# Autodesk Inventor assembly: BBM - Simplified
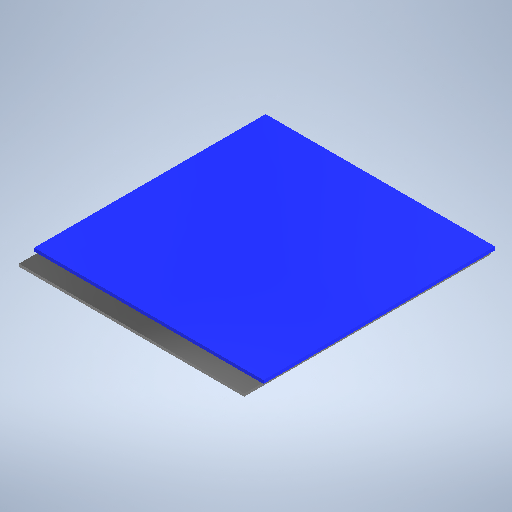
[picture p0: Inventor's stored thumbnail of the model, 512x512]
Saved by Autodesk Inventor 2025 (Build 290162000, 162)
## iProperties
Created: 2022-02-01
Part Number: BBM - Simplified
Document SubType Name: Assembly
Designer: Caleb
Author: Caleb
## Documents named in this file (4)
- C:\Users\cfang\Desktop\nebraska-silicon-lab\Hardware\ETL\modules\Tamale v1.6\BBM - Simplified.iam
- C:\Users\cfang\Desktop\nebraska-silicon-lab\Hardware\ETL\modules\Tamale v1.6\ETL Sensor.ipt
- C:\Users\cfang\Desktop\nebraska-silicon-lab\Hardware\ETL\modules\Tamale v1.6\bump bond.ipt
- C:\Users\cfang\Desktop\nebraska-silicon-lab\Hardware\ETL\modules\Tamale v1.6\ETROC2 - Simplified.ipt
## Components (3 placed, 3 different names)
1. ETL Sensor:1 — Tangent:1, Tangent:2, Tangent:3, Flush:1, Flush:2, Mate:1
2. bump bond:1 — Tangent:1, Tangent:2, Tangent:3
3. ETROC2 - Simplified:1 — Flush:1, Flush:2, Mate:1
## Relationships (6: Tangent 3, Flush 2, Mate 1)
- Tangent:1: ETL Sensor:1 ↔ bump bond:1
- Tangent:2 (-0.65 mm): ETL Sensor:1 ↔ bump bond:1
- Tangent:3 (-0.65 mm): ETL Sensor:1 ↔ bump bond:1
- Flush:1 (0.2 mm): ETL Sensor:1 ↔ ETROC2 - Simplified:1
- Flush:2 (0.2 mm): ETL Sensor:1 ↔ ETROC2 - Simplified:1
- Mate:1 (0.08 mm): ETL Sensor:1 ↔ ETROC2 - Simplified:1
